# Autodesk Inventor assembly: Burning Table Assembly
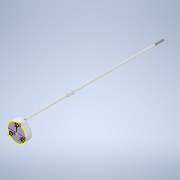
[picture p0: Inventor's stored thumbnail of the model, 180x180]
Saved by Autodesk Inventor 2020 (Build 240168000, 168)
## iProperties
Created: 2019-06-07
Part Number: Burning Table Assembly
Document SubType Name: Assembly
Designer: isadmin
Author: isadmin
## Documents named in this file (3)
- C:\Users\ColinP\Documents\Inventor\INVENTOR IS_2019June01\Burning Table Assembly.iam
- C:\Users\ColinP\Documents\Inventor\INVENTOR IS_2019June01\Burner Table IS v01.ipt
- C:\Users\ColinP\Documents\Inventor\igor\assembly of 13 and 2.iam
## Components (2 placed, 2 different names)
1. Burner Table IS v01:1 — Insert:1
2. assembly of 13 and 2:1 [sub-assembly] — Insert:1
## Relationships (1: Insert 1)
- Insert:1: Burner Table IS v01:1 ↔ assembly of 13 and 2:1
